# Autodesk Inventor assembly: BEC_Assembly
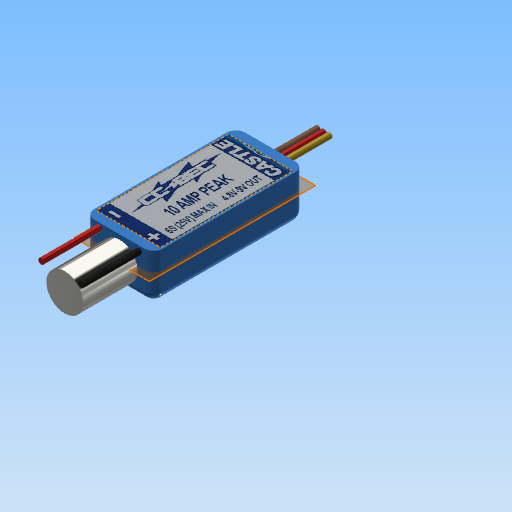
[picture p0: Inventor's stored thumbnail of the model, 512x512]
Saved by Autodesk Inventor 2017 (Build 210142000, 142)
## iProperties
Created: 2017-05-21
Part Number: BEC_Assembly
Document SubType Name: Assembly
Designer: Derek Wider
Author: Derek Wider
## Documents named in this file (7)
- E:\OneDrive\Documents\Other Projects\Submarine\CAD\midships\ElectronicsSection\BEC\BEC_Assembly.iam
- E:\OneDrive\Documents\Other Projects\Submarine\CAD\midships\ElectronicsSection\BEC\BEC_CAP.ipt
- E:\OneDrive\Documents\Other Projects\Submarine\CAD\midships\ElectronicsSection\BEC\Body.ipt
- E:\OneDrive\Documents\Other Projects\Submarine\CAD\midships\ElectronicsSection\BEC\Wire_Black.ipt
- E:\OneDrive\Documents\Other Projects\Submarine\CAD\midships\ElectronicsSection\BEC\Wire_Brown.ipt
- E:\OneDrive\Documents\Other Projects\Submarine\CAD\midships\ElectronicsSection\BEC\Wire_Red.ipt
- E:\OneDrive\Documents\Other Projects\Submarine\CAD\midships\ElectronicsSection\BEC\Wire_Yellow.ipt
## Components (7 placed, 6 different names)
1. Body:1 — Tangent:1, Tangent:2, Mate:1, Mate:2, Mate:3, Flush:1, Mate:7, Mate:8
2. BEC_CAP:2 — Tangent:1, Tangent:2
3. Wire_Black:1 — Mate:7
4. Wire_Brown:1 — Tangent:3, Mate:1, Mate:6
5. Wire_Red:1 — Tangent:3, Tangent:4, Mate:2, Mate:5
6. Wire_Yellow:1 — Tangent:4, Mate:3, Mate:4
7. Wire_Red:2 — Mate:8
## Relationships (13: Mate 8, Tangent 4, Flush 1)
- Tangent:1 (1 mm): Body:1 ↔ BEC_CAP:2
- Tangent:2 (1.5 mm): Body:1 ↔ BEC_CAP:2
- Tangent:3: Wire_Brown:1 ↔ Wire_Red:1
- Tangent:4: Wire_Red:1 ↔ Wire_Yellow:1
- Mate:1: Body:1 ↔ Wire_Brown:1
- Mate:2: Body:1 ↔ Wire_Red:1
- Mate:3: Body:1 ↔ Wire_Yellow:1
- Flush:1 (-4 mm): Body:1
- Mate:4: Wire_Yellow:1
- Mate:5: Wire_Red:1
- Mate:6: Wire_Brown:1
- Mate:7: Body:1 ↔ Wire_Black:1
- Mate:8: Body:1 ↔ Wire_Red:2
